# Autodesk Inventor assembly: wooden
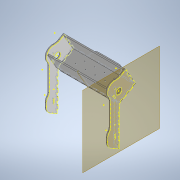
[picture p0: Inventor's stored thumbnail of the model, 180x180]
Saved by Autodesk Inventor 2020 (Build 240168000, 168)
## iProperties
Created: 2019-07-24
Part Number: wooden
Document SubType Name: Assembly
Designer: erwin
Author: erwin
## Documents named in this file (5)
- D:\GitHub\BeachMaid\platform\wooden_assembly.iam
- D:\GitHub\BeachMaid\platform\wooden_side.ipt
- D:\GitHub\BeachMaid\platform\wooden_lip.ipt
- D:\GitHub\BeachMaid\platform\wooden_back.ipt
- D:\GitHub\BeachMaid\platform\dxf\wooden_bottom.ipt
## Components (5 placed, 4 different names)
1. wooden_side:1 — Flush:1, Flush:2, Flush:3, Flush:4, Flush:5, Flush:6, Flush:7, Flush:8, Flush:9, Flush:10, Flush:11, Flush:12
2. wooden_lip:1 — Flush:1, Flush:2, Flush:3, Flush:13
3. wooden_back:1 — Flush:4, Flush:5, Flush:6, Flush:7, Flush:14
4. wooden_bottom:1 — Flush:8, Flush:9, Flush:10, Flush:11, Flush:12, Flush:15
5. wooden_side:2 — Flush:13, Flush:14, Flush:15
## Relationships (15: Flush 15)
- Flush:1: wooden_side:1 ↔ wooden_lip:1
- Flush:2: wooden_side:1 ↔ wooden_lip:1
- Flush:3: wooden_side:1 ↔ wooden_lip:1
- Flush:4: wooden_side:1 ↔ wooden_back:1
- Flush:5: wooden_side:1 ↔ wooden_back:1
- Flush:6: wooden_side:1 ↔ wooden_back:1
- Flush:7: wooden_side:1 ↔ wooden_back:1
- Flush:8: wooden_side:1 ↔ wooden_bottom:1
- Flush:9: wooden_side:1 ↔ wooden_bottom:1
- Flush:10: wooden_side:1 ↔ wooden_bottom:1
- Flush:11: wooden_side:1 ↔ wooden_bottom:1
- Flush:12: wooden_side:1 ↔ wooden_bottom:1
- Flush:13: wooden_lip:1 ↔ wooden_side:2
- Flush:14: wooden_back:1 ↔ wooden_side:2
- Flush:15: wooden_bottom:1 ↔ wooden_side:2
